# Autodesk Inventor assembly: Assembly2
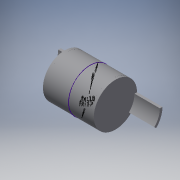
[picture p0: Inventor's stored thumbnail of the model, 180x180]
Saved by Autodesk Inventor 2019 (Build 230136000, 136)
## iProperties
Created: 2018-07-17
Part Number: Assembly2
Document SubType Name: Assembly
Designer: Ge Shi
Author: Ge Shi
## Documents named in this file (5)
- D:\hive\projects\knee-patella\Assembly2.iam
- D:\hive\projects\knee-patella\knee ball.ipt
- D:\hive\projects\knee-patella\lower leg V2.ipt
- D:\hive\projects\knee-patella\upper leg V2.ipt
- D:\hive\projects\knee-patella\custom support at hinge V2.ipt
## Components (4 placed, 4 different names)
1. knee ball:1 — Mate:3
2. lower leg V2:1 — Mate:3, Mate:5, Mate:6, Flush:1, Mate:8, Mate:9
3. upper leg V2:1 — Mate:5, Mate:6, Flush:1, Mate:7
4. custom support at hinge V2:1 — Mate:7, Mate:8, Mate:9
## Relationships (7: Mate 6, Flush 1)
- Mate:3: knee ball:1 ↔ lower leg V2:1
- Mate:5 (1 mm): lower leg V2:1 ↔ upper leg V2:1
- Mate:6: lower leg V2:1 ↔ upper leg V2:1
- Flush:1: lower leg V2:1 ↔ upper leg V2:1
- Mate:7: upper leg V2:1 ↔ custom support at hinge V2:1
- Mate:8: lower leg V2:1 ↔ custom support at hinge V2:1
- Mate:9: lower leg V2:1 ↔ custom support at hinge V2:1
## Named parameters: clearance = 1 mm
